# Autodesk Inventor assembly: Wheel
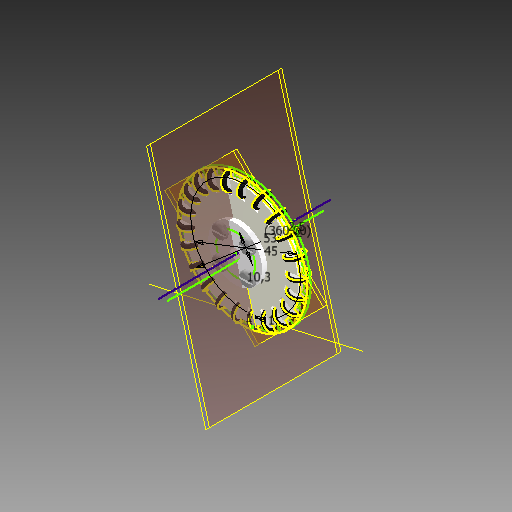
[picture p0: Inventor's stored thumbnail of the model, 512x512]
Saved by Autodesk Inventor 2020 (Build 240168000, 168)
## iProperties
Created: 2024-10-05
Part Number: Wheel
Document SubType Name: Assembly
Designer: Ivan
Mass: 7.4683 g
Surface Area: 125.902 cm^2
Volume: 7.4683 cm^3
Density: 1 g/cm^3
Author: Ivan
## Documents named in this file (8)
- C:\!projects\DASH-\3D\Dash-V1\wheel\Wheel.iam
- C:\!projects\DASH-\3D\Dash-V1\wheel\wheel_board.ipt
- C:\!projects\DASH-\3D\Dash-V1\wheel\wheel_ring.ipt
- C:\!projects\DASH-\3D\Dash-V1\wheel\sub_wheel.ipt
- C:\!projects\DASH-\3D\Dash-V1\wheel\wheel_board_ЗЕРКАЛО.ipt
- C:\!projects\DASH-\3D\Dash-V1\step\4mm Rigid Flange Coupling v2.iam
- C:\!projects\DASH-\3D\Dash-V1\step\m3_bolt\m3x8\Винт А.М3-6gx8 ГОСТ 11644-75.ipt
- C:\!projects\DASH-\3D\Dash-V1\step\m3_bolt\m3x8\Гайка М3-6H ГОСТ 5927-70.ipt
## Components (34 placed, 7 different names)
1. wheel_board:1 — Совмещение:1, Совмещение:2, Заподлицо:1, Совмещение:3, Совмещение:4, Вставка:7, Вставка:8, Вставка:9, Вставка:10
2. wheel_ring:1 — Заподлицо:2, Заподлицо:3
3. wheel_board_ЗЕРКАЛО:1 — Совмещение:5, Совмещение:6, Совмещение:7, Совмещение:8, Вставка:1, Вставка:2
4. 4mm Rigid Flange Coupling v2:1 [sub-assembly] — Вставка:1, Вставка:2, Вставка:3, Вставка:4, Вставка:5, Вставка:6
5. Винт А.М3-6gx8 ГОСТ 11644-75:1 — Вставка:3
6. Винт А.М3-6gx8 ГОСТ 11644-75:2 — Вставка:5
7. Винт А.М3-6gx8 ГОСТ 11644-75:3 — Вставка:6
8. Винт А.М3-6gx8 ГОСТ 11644-75:4 — Вставка:4
9. Гайка М3-6H ГОСТ 5927-70:1 — Вставка:10
10. Гайка М3-6H ГОСТ 5927-70:2 — Вставка:9
11. Гайка М3-6H ГОСТ 5927-70:3 — Вставка:8
12. Гайка М3-6H ГОСТ 5927-70:4 — Вставка:7
13. sub_wheel:1 — Совмещение:3
14. sub_wheel:2
15. sub_wheel:3
16. sub_wheel:4
17. sub_wheel:5
18. sub_wheel:6
19. sub_wheel:7
20. sub_wheel:8
21. sub_wheel:9
22. sub_wheel:10
23. sub_wheel:11
24. sub_wheel:12
25. sub_wheel:13
26. sub_wheel:14
27. sub_wheel:15
28. sub_wheel:16
29. sub_wheel:17
30. sub_wheel:18
31. sub_wheel:19
32. sub_wheel:20
33. sub_wheel:21
34. sub_wheel:22
## Component patterns: (22 elements, first: sub_wheel:1)
## Relationships (21: Insert 10, Mate 8, Flush 3)
- Совмещение:1 [Mate]: wheel_board:1
- Совмещение:2 [Mate]: wheel_board:1
- Заподлицо:1 [Flush]: wheel_board:1
- Заподлицо:2 [Flush]: wheel_ring:1
- Заподлицо:3 [Flush]: wheel_ring:1
- Совмещение:3 [Mate] (0.05 mm): wheel_board:1 ↔ sub_wheel:1
- Совмещение:4 [Mate]: wheel_board:1
- Совмещение:5 [Mate]: wheel_board_ЗЕРКАЛО:1
- Совмещение:6 [Mate]: wheel_board_ЗЕРКАЛО:1
- Совмещение:7 [Mate]: wheel_board_ЗЕРКАЛО:1
- Совмещение:8 [Mate]: wheel_board_ЗЕРКАЛО:1
- Вставка:1 [Insert]: wheel_board_ЗЕРКАЛО:1 ↔ 4mm Rigid Flange Coupling v2:1
- Вставка:2 [Insert]: wheel_board_ЗЕРКАЛО:1 ↔ 4mm Rigid Flange Coupling v2:1
- Вставка:3 [Insert]: 4mm Rigid Flange Coupling v2:1 ↔ Винт А.М3-6gx8 ГОСТ 11644-75:1
- Вставка:4 [Insert]: 4mm Rigid Flange Coupling v2:1 ↔ Винт А.М3-6gx8 ГОСТ 11644-75:4
- Вставка:5 [Insert]: 4mm Rigid Flange Coupling v2:1 ↔ Винт А.М3-6gx8 ГОСТ 11644-75:2
- Вставка:6 [Insert]: 4mm Rigid Flange Coupling v2:1 ↔ Винт А.М3-6gx8 ГОСТ 11644-75:3
- Вставка:7 [Insert]: wheel_board:1 ↔ Гайка М3-6H ГОСТ 5927-70:4
- Вставка:8 [Insert]: wheel_board:1 ↔ Гайка М3-6H ГОСТ 5927-70:3
- Вставка:9 [Insert]: wheel_board:1 ↔ Гайка М3-6H ГОСТ 5927-70:2
- Вставка:10 [Insert]: wheel_board:1 ↔ Гайка М3-6H ГОСТ 5927-70:1
